# Autodesk Inventor assembly: Floor_System
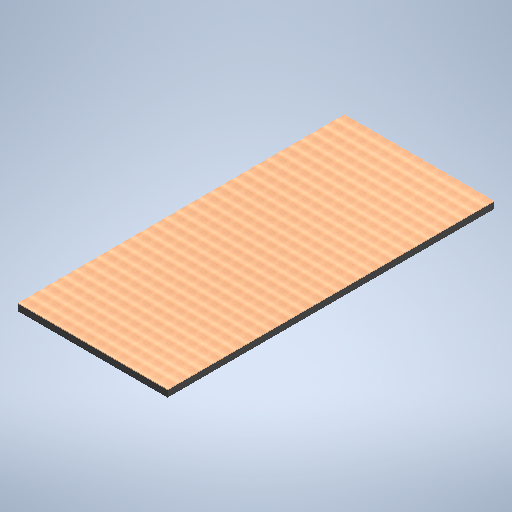
[picture p0: Inventor's stored thumbnail of the model, 512x512]
Saved by Autodesk Inventor 2025 (Build 290162010, 162A)
## iProperties
Created: 2024-09-15
Part Number: Floor_System
Document SubType Name: Assembly
Designer: Tom
Author: Tom
## Documents named in this file (6)
- C:\Users\Tom\Documents\Inventor\Mobility\Additional_Building\Floor_System.iam
- C:\Users\Tom\Documents\Inventor\Mobility\Additional_Building\Beam.iam
- C:\Users\Tom\Documents\Inventor\Mobility\Additional_Building\Joist_With_Length_56.5625_Inches.iam
- C:\Users\Tom\Documents\Inventor\Mobility\Additional_Building\Joist_With_Length_6.375_Inches.iam
- C:\Users\Tom\Documents\Inventor\Mobility\Additional_Building\Joist_With_Length_144_Inches.iam
- C:\Users\Tom\Documents\Inventor\Mobility\Additional_Building\Subfloor.ipt
## Components (66 placed, 5 different names)
1. Subfloor:1 — Mate:4, Flush:7, Flush:8
2. Beam:1 [sub-assembly] — Mate:2, Flush:3, Flush:4
3. Beam:2 [sub-assembly]
4. Beam:3 [sub-assembly]
5. Beam:4 [sub-assembly]
6. Beam:5 [sub-assembly] — Mate:1, Flush:1, Flush:2
7. Beam:6 [sub-assembly]
8. Joist_With_Length_56.5625_Inches:1 [sub-assembly] — Mate:1, Flush:1, Flush:2
9. Joist_With_Length_56.5625_Inches:2 [sub-assembly]
10. Joist_With_Length_56.5625_Inches:3 [sub-assembly]
11. Joist_With_Length_56.5625_Inches:4 [sub-assembly]
12. Joist_With_Length_56.5625_Inches:5 [sub-assembly]
13. Joist_With_Length_56.5625_Inches:6 [sub-assembly]
14. Joist_With_Length_56.5625_Inches:7 [sub-assembly]
15. Joist_With_Length_56.5625_Inches:8 [sub-assembly]
16. Joist_With_Length_56.5625_Inches:9 [sub-assembly]
17. Joist_With_Length_56.5625_Inches:10 [sub-assembly]
18. Joist_With_Length_56.5625_Inches:11 [sub-assembly]
19. Joist_With_Length_56.5625_Inches:12 [sub-assembly]
20. Joist_With_Length_56.5625_Inches:13 [sub-assembly]
21. Joist_With_Length_56.5625_Inches:14 [sub-assembly]
22. Joist_With_Length_56.5625_Inches:15 [sub-assembly]
23. Joist_With_Length_56.5625_Inches:16 [sub-assembly]
24. Joist_With_Length_56.5625_Inches:17 [sub-assembly]
25. Joist_With_Length_56.5625_Inches:18 [sub-assembly]
26. Joist_With_Length_56.5625_Inches:19 [sub-assembly]
27. Joist_With_Length_56.5625_Inches:20 [sub-assembly]
28. Joist_With_Length_56.5625_Inches:21 [sub-assembly]
29. Joist_With_Length_56.5625_Inches:22 [sub-assembly]
30. Joist_With_Length_56.5625_Inches:23 [sub-assembly]
31. Joist_With_Length_56.5625_Inches:24 [sub-assembly]
32. Joist_With_Length_56.5625_Inches:25 [sub-assembly]
33. Joist_With_Length_56.5625_Inches:26 [sub-assembly]
34. Joist_With_Length_56.5625_Inches:27 [sub-assembly]
35. Joist_With_Length_56.5625_Inches:28 [sub-assembly]
36. Joist_With_Length_56.5625_Inches:29 [sub-assembly]
37. Joist_With_Length_56.5625_Inches:30 [sub-assembly]
38. Joist_With_Length_56.5625_Inches:31 [sub-assembly]
39. Joist_With_Length_56.5625_Inches:32 [sub-assembly]
40. Joist_With_Length_56.5625_Inches:33 [sub-assembly]
41. Joist_With_Length_56.5625_Inches:34 [sub-assembly]
42. Joist_With_Length_56.5625_Inches:35 [sub-assembly]
43. Joist_With_Length_56.5625_Inches:36 [sub-assembly]
44. Joist_With_Length_56.5625_Inches:37 [sub-assembly]
45. Joist_With_Length_56.5625_Inches:38 [sub-assembly] — Flush:8
46. Joist_With_Length_6.375_Inches:1 [sub-assembly] — Mate:2, Flush:3, Flush:4, Mate:3, Flush:5, Flush:6
47. Joist_With_Length_6.375_Inches:2 [sub-assembly]
48. Joist_With_Length_6.375_Inches:3 [sub-assembly]
49. Joist_With_Length_6.375_Inches:4 [sub-assembly]
50. Joist_With_Length_6.375_Inches:5 [sub-assembly]
51. Joist_With_Length_6.375_Inches:6 [sub-assembly]
52. Joist_With_Length_6.375_Inches:7 [sub-assembly]
53. Joist_With_Length_6.375_Inches:8 [sub-assembly]
54. Joist_With_Length_6.375_Inches:9 [sub-assembly]
55. Joist_With_Length_6.375_Inches:10 [sub-assembly]
56. Joist_With_Length_6.375_Inches:11 [sub-assembly]
57. Joist_With_Length_6.375_Inches:12 [sub-assembly]
58. Joist_With_Length_6.375_Inches:13 [sub-assembly]
59. Joist_With_Length_6.375_Inches:14 [sub-assembly]
60. Joist_With_Length_6.375_Inches:15 [sub-assembly]
61. Joist_With_Length_6.375_Inches:16 [sub-assembly]
62. Joist_With_Length_6.375_Inches:17 [sub-assembly]
63. Joist_With_Length_6.375_Inches:18 [sub-assembly]
64. Joist_With_Length_6.375_Inches:19 [sub-assembly]
65. Joist_With_Length_144_Inches:1 [sub-assembly] — Mate:3, Flush:5, Flush:6
66. Joist_With_Length_144_Inches:2 [sub-assembly] — Mate:4, Flush:7
## Component patterns: (6 elements, first: Beam:1), (38 elements, first: Joist_With_Length_56.5625_Inches:1), (19 elements, first: Joist_With_Length_6.375_Inches:1), (2 elements, first: Joist_With_Length_144_Inches:1)
## Relationships (12: Flush 8, Mate 4)
- Mate:1: Beam:5 ↔ Joist_With_Length_56.5625_Inches:1
- Flush:1: Beam:5 ↔ Joist_With_Length_56.5625_Inches:1
- Flush:2: Beam:5 ↔ Joist_With_Length_56.5625_Inches:1
- Mate:2: Beam:1 ↔ Joist_With_Length_6.375_Inches:1
- Flush:3: Beam:1 ↔ Joist_With_Length_6.375_Inches:1
- Flush:4: Beam:1 ↔ Joist_With_Length_6.375_Inches:1
- Mate:3: Joist_With_Length_6.375_Inches:1 ↔ Joist_With_Length_144_Inches:1
- Flush:5: Joist_With_Length_6.375_Inches:1 ↔ Joist_With_Length_144_Inches:1
- Flush:6: Joist_With_Length_6.375_Inches:1 ↔ Joist_With_Length_144_Inches:1
- Mate:4: Subfloor:1 ↔ Joist_With_Length_144_Inches:2
- Flush:7: Subfloor:1 ↔ Joist_With_Length_144_Inches:2
- Flush:8: Subfloor:1 ↔ Joist_With_Length_56.5625_Inches:38
